# Autodesk Inventor assembly: Double Acting Piston With Hardware
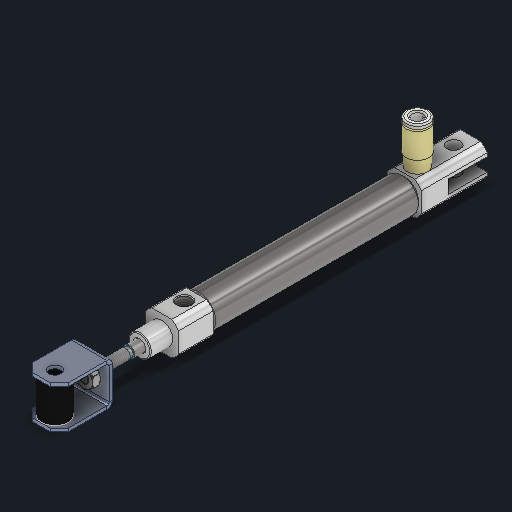
[picture p0: Inventor's stored thumbnail of the model, 512x512]
Saved by Autodesk Inventor 2025.1 (Build 291241000, 241)
## iProperties
Created: 2022-09-23
Part Number: Double Acting Piston With Hardware
Document SubType Name: Assembly
Designer: maxxw
Mass: 9.29214 g
Surface Area: 91.0706 cm^2
Volume: 9.29214 cm^3
Density: 1 g/cm^3
Author: maxxw
## Documents named in this file (8)
- C:\Users\avere\VEX\High Stakes\CAD\ROBOPROS-CAD-Inventor\Motion\Pneumatics\Double Acting Piston With Hardware.iam
- C:\Users\avere\VEX\High Stakes\CAD\ROBOPROS-CAD-Inventor\Motion\Pneumatics\Reference Parts\Pistons\Double Acting Piston Body.ipt
- C:\Users\avere\VEX\High Stakes\CAD\ROBOPROS-CAD-Inventor\Motion\Pneumatics\Reference Parts\Pistons\Double Acting Piston Rod.ipt
- C:\Users\avere\VEX\High Stakes\CAD\ROBOPROS-CAD-Inventor\Structure\Hardware\Nut Hex #6-32.ipt
- C:\Users\avere\VEX\High Stakes\CAD\ROBOPROS-CAD-Inventor\Motion\Pneumatics\Cylinder Mount.ipt
- C:\Users\avere\VEX\High Stakes\CAD\ROBOPROS-CAD-Inventor\Motion\Pneumatics\Fitting for Cylinders.ipt
- C:\Users\avere\VEX\High Stakes\CAD\ROBOPROS-CAD-Inventor\Motion\Spacers\Spacer Nylon .375 OD\NSpacer .375 OD x .500.ipt
- C:\Users\avere\VEX\High Stakes\CAD\ROBOPROS-CAD-Inventor\Motion\Spacers\Spacer Nylon .375 OD.ipt
## Components (7 placed, 6 different names)
1. Double Acting Piston Body:1 — Mate:1, Mate:2, Insert:4
2. Double Acting Piston Rod:1 — Mate:1, Mate:2, Insert:3
3. Nut Hex #6-32:1 — Insert:1, Insert:3
4. Nut Hex #6-32:2 — Insert:2
5. Cylinder Mount:1 — Insert:1, Insert:2, Insert:5
6. Fitting for Cylinders:1 — Insert:4
7. NSpacer .375 OD x .500:1 — Insert:5
## Relationships (7: Insert 5, Mate 2)
- Mate:1: Double Acting Piston Body:1 ↔ Double Acting Piston Rod:1
- Mate:2: Double Acting Piston Body:1 ↔ Double Acting Piston Rod:1
- Insert:1: Nut Hex #6-32:1 ↔ Cylinder Mount:1
- Insert:2: Nut Hex #6-32:2 ↔ Cylinder Mount:1
- Insert:3: Double Acting Piston Rod:1 ↔ Nut Hex #6-32:1
- Insert:4: Double Acting Piston Body:1 ↔ Fitting for Cylinders:1
- Insert:5: Cylinder Mount:1 ↔ NSpacer .375 OD x .500:1
